# Autodesk Inventor assembly: M178-3000
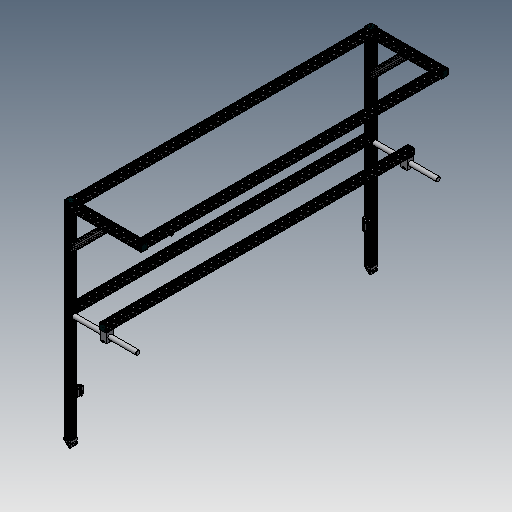
[picture p0: Inventor's stored thumbnail of the model, 512x512]
Saved by Autodesk Inventor 2018.3 (Build 223284000, 284)
## iProperties
Created: 2004-11-23
Part Number: M178-3000
Document SubType Name: Assembly
Designer: Autodesk, Inc.
Manufacturer: Standard
Standards Organization: Custom
Mass: 21755.3 g
Surface Area: 53805.5 cm^2
Volume: 7961.35 cm^3
Density: 2.73262 g/cm^3
CAGE: 1LJX3
Dept. ID: Product Design
Description #2: ---
Finish #1: ---
Finish #2: ---
Material ID: ---
Project Number: ---
Author: Autodesk, Inc.
## Documents named in this file (13)
- C:\AVAInvAPI\Workspace\Test Station\Components\M178-3000.iam
- C:\AVAInvAPI\Workspace\Test Station\Components\M178-3001.ipt
- C:\AVAInvAPI\Workspace\Test Station\Components\21-135 Corner Phantom.iam
- C:\AVAInvAPI\Workspace\Test Station\Components\21-135 Corner Phantom 2.iam
- C:\AVAInvAPI\Workspace\Test Station\Components\M178-3002.ipt
- C:\AVAInvAPI\Workspace\Test Station\Components\M178-100_Cross_Phantom.iam
- C:\AVAInvAPI\Workspace\Test Station\Components\M178-3000 Overhange Phantom.iam
- C:\AVAInvAPI\Workspace\Test Station\Components\22-136.ipt
- C:\AVAInvAPI\Workspace\Test Station\Components\22-130.iam
- C:\AVAInvAPI\Workspace\Test Station\Components\18-813.ipt
- C:\AVAInvAPI\Workspace\Test Station\Components\22-134.iam
- C:\Users\kelleyb.ADS\Desktop\Samples MIGRATED 2009 224 RTM_1\Standard Parts\Test Station Content\Extrusions\40 Series Profiles.ipt
- C:\Users\kelleyb.ADS\Desktop\Samples MIGRATED 2009 224 RTM_1\Standard Parts\Test Station Content\End Caps\18-xxx 40 Series End Caps.ipt
## Components (23 placed, 10 different names)
1. M178-3001:1 — Flush:1, Mate:1, Flush:3, Flush:4, Mate:4, Mate:5, Flush:6, Mate:6, Angle:1, Flush:7, Mate:8, Mate:9, Mate:10, Flush:11, Mate:13, Flush:12, Flush:13, Mate:14, Flush:14, Flush:15, Insert:2, Angle:3
2. M178-3001:2 — Mate:1, Flush:3, Flush:4, Mate:7, Flush:9
3. 21-135 Corner Phantom:1 [sub-assembly] — Mate:6, Angle:1, Flush:7, Flush:10
4. 21-135 Corner Phantom:2 [sub-assembly] — Mate:7, Flush:9, Flush:10
5. M178-3002:3 — Mate:11, Flush:11, Mate:12, Insert:4, Angle:4, Insert:5, Angle:5
6. M178-100_Cross_Phantom:3 [sub-assembly] — Mate:15, Flush:16, Flush:17, Mate:16, Flush:18
7. 22-136:1 — Mate:16, Flush:18
8. 18-813:5 — Insert:4, Angle:4
9. 18-813:6 — Insert:5, Angle:5
10. 22-130:1 [sub-assembly] — Mate:8, Mate:9, Mate:10, Insert:1
11. 22-134:1 [sub-assembly] — Mate:11, Mate:12, Insert:1
12. 22-130:2 [sub-assembly]
13. 22-134:2 [sub-assembly]
14. 21-135 Corner Phantom 2:1 [sub-assembly] — Mate:4, Mate:5, Flush:6
15. 21-135 Corner Phantom 2:2 [sub-assembly]
16. M178-100_Cross_Phantom:1 [sub-assembly] — Mate:13, Flush:12, Flush:13
17. M178-100_Cross_Phantom:2 [sub-assembly]
18. M178-3000 Overhange Phantom:1 [sub-assembly] — Mate:14, Flush:14, Flush:15, Mate:15, Flush:16, Flush:17, Insert:3, Angle:2
19. 18-813:1 — Insert:2, Angle:3
20. 18-813:2 — Insert:3, Angle:2
21. M178-3000 Overhange Phantom:2 [sub-assembly]
22. 18-813:7
23. 18-813:8
## Component patterns: (2 elements, first: 22-130:1 + 22-134:1), (2 elements, first: 21-135 Corner Phantom 2:1), (2 elements, first: M178-100_Cross_Phantom:1), (2 elements, first: M178-3000 Overhange Phantom:1 + 18-813:1 + 18-813:2)
## Relationships (42: Flush 17, Mate 15, Angle 5, Insert 5)
- Flush:1 (-914.4 mm): M178-3001:1
- Mate:1 (-1828.8 mm): M178-3001:1 ↔ M178-3001:2
- Flush:3: M178-3001:1 ↔ M178-3001:2
- Flush:4: M178-3001:1 ↔ M178-3001:2
- [Mate]: M178-3001:1
- [Flush]: M178-3001:1
- Mate:4: M178-3001:1 ↔ 21-135 Corner Phantom 2:1
- Mate:5: M178-3001:1 ↔ 21-135 Corner Phantom 2:1
- Flush:6: M178-3001:1 ↔ 21-135 Corner Phantom 2:1
- Mate:6: M178-3001:1 ↔ 21-135 Corner Phantom:1
- Angle:1 (0 deg): M178-3001:1 ↔ 21-135 Corner Phantom:1
- Flush:7: M178-3001:1 ↔ 21-135 Corner Phantom:1
- [Flush] (203.2 mm): M178-3001:1 ↔ 21-135 Corner Phantom:1
- Mate:7: M178-3001:2 ↔ 21-135 Corner Phantom:2
- Flush:9: M178-3001:2 ↔ 21-135 Corner Phantom:2
- Flush:10: 21-135 Corner Phantom:1 ↔ 21-135 Corner Phantom:2
- Mate:8: M178-3001:1 ↔ 22-130:1
- Mate:9: M178-3001:1 ↔ 22-130:1
- Mate:10 (-635 mm): M178-3001:1 ↔ 22-130:1
- Mate:11: M178-3002:3 ↔ 22-134:1
- Flush:11: M178-3001:1 ↔ M178-3002:3
- Mate:12: M178-3002:3 ↔ 22-134:1
- Mate:13: M178-3001:1 ↔ M178-100_Cross_Phantom:1
- Flush:12: M178-3001:1 ↔ M178-100_Cross_Phantom:1
- Flush:13 (635 mm): M178-3001:1 ↔ M178-100_Cross_Phantom:1
- Insert:1 (-203.2 mm): 22-130:1 ↔ 22-134:1
- Mate:14: M178-3001:1 ↔ M178-3000 Overhange Phantom:1
- Flush:14: M178-3001:1 ↔ M178-3000 Overhange Phantom:1
- Flush:15: M178-3001:1 ↔ M178-3000 Overhange Phantom:1
- Mate:15: M178-100_Cross_Phantom:3 ↔ M178-3000 Overhange Phantom:1
- Flush:16: M178-100_Cross_Phantom:3 ↔ M178-3000 Overhange Phantom:1
- Flush:17: M178-100_Cross_Phantom:3 ↔ M178-3000 Overhange Phantom:1
- Mate:16: M178-100_Cross_Phantom:3 ↔ 22-136:1
- Flush:18: M178-100_Cross_Phantom:3 ↔ 22-136:1
- Insert:2: M178-3001:1 ↔ 18-813:1
- Insert:3: M178-3000 Overhange Phantom:1 ↔ 18-813:2
- Angle:2 (0 deg): M178-3000 Overhange Phantom:1 ↔ 18-813:2
- Angle:3 (0 deg): M178-3001:1 ↔ 18-813:1
- Insert:4: M178-3002:3 ↔ 18-813:5
- Angle:4 (0 deg): M178-3002:3 ↔ 18-813:5
- Insert:5: M178-3002:3 ↔ 18-813:6
- Angle:5 (0 deg): M178-3002:3 ↔ 18-813:6
